# Autodesk Inventor assembly: ASDSAssembly
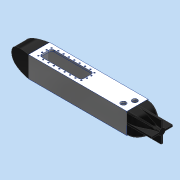
[picture p0: Inventor's stored thumbnail of the model, 180x180]
Saved by Autodesk Inventor 2018 (Build 220112000, 112)
## iProperties
Created: 2017-02-12
Part Number: ASDSAssembly
Document SubType Name: Assembly
Designer: techn
Author: techn
## Documents named in this file (5)
- D:\Projects\Submarine-project\CAD\ASDS\ASDSAssembly.iam
- D:\Projects\Submarine-project\CAD\ASDS\Fore.ipt
- D:\Projects\Submarine-project\CAD\ASDS\Aft.ipt
- D:\Projects\Submarine-project\CAD\ASDS\Hull_Alu.ipt
- D:\Projects\Submarine-project\CAD\ASDS\ForeAftMountPlate.ipt
## Components (5 placed, 4 different names)
1. Fore:1 — Mate:1, Mate:2, Mate:3, Mate:7, Mate:8, Mate:9
2. Hull_Alu:1 — Mate:1, Mate:2, Mate:3, Mate:4, Mate:5, Mate:6
3. Aft:1 — Mate:4, Mate:5, Mate:6, Mate:10, Mate:11, Mate:12
4. ForeAftMountPlate:1 — Mate:7, Mate:8, Mate:9
5. ForeAftMountPlate:2 — Mate:10, Mate:11, Mate:12
## Relationships (12: Mate 12)
- Mate:1: Fore:1 ↔ Hull_Alu:1
- Mate:2: Fore:1 ↔ Hull_Alu:1
- Mate:3: Fore:1 ↔ Hull_Alu:1
- Mate:4: Hull_Alu:1 ↔ Aft:1
- Mate:5: Hull_Alu:1 ↔ Aft:1
- Mate:6: Hull_Alu:1 ↔ Aft:1
- Mate:7: Fore:1 ↔ ForeAftMountPlate:1
- Mate:8: Fore:1 ↔ ForeAftMountPlate:1
- Mate:9: Fore:1 ↔ ForeAftMountPlate:1
- Mate:10: Aft:1 ↔ ForeAftMountPlate:2
- Mate:11: Aft:1 ↔ ForeAftMountPlate:2
- Mate:12: Aft:1 ↔ ForeAftMountPlate:2
